# Autodesk Inventor assembly: borde dos piezas
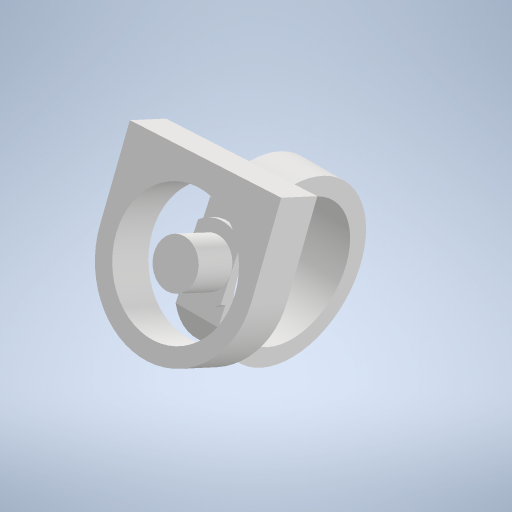
[picture p0: Inventor's stored thumbnail of the model, 512x512]
Saved by Autodesk Inventor 2024 (Build 280153000, 153)
## iProperties
Created: 2024-04-03
Part Number: borde dos piezas
Document SubType Name: Assembly
Designer: compu
Author: compu
## Documents named in this file (3)
- C:\Users\compu\Documents\1Juan\1Facultad\9 Semestre\E1225 Taller de Sistemas Digitales\Parts\borde dos piezas\borde dos piezas.iam
- C:\Users\compu\Documents\1Juan\1Facultad\9 Semestre\E1225 Taller de Sistemas Digitales\Parts\borde dos piezas\borde al borde.ipt
- C:\Users\compu\Documents\1Juan\1Facultad\9 Semestre\E1225 Taller de Sistemas Digitales\Parts\borde dos piezas\borde libre.ipt
## Components (2 placed, 2 different names)
1. borde al borde:1 — Insert:1
2. borde libre:1 — Mate:1, Insert:1, Flush:1
## Relationships (3: Mate 1, Insert 1, Flush 1)
- Mate:1: borde libre:1
- Insert:1: borde al borde:1 ↔ borde libre:1
- Flush:1: borde libre:1
